# Autodesk Inventor assembly: face
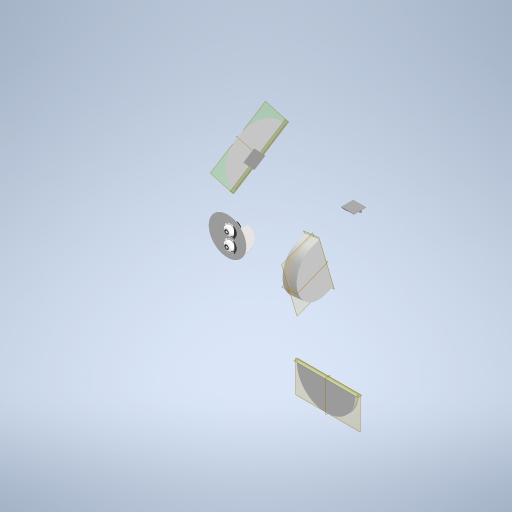
[picture p0: Inventor's stored thumbnail of the model, 512x512]
Saved by Autodesk Inventor 2023.2 (Build 272271030, 271C)
## iProperties
Created: 2024-01-26
Part Number: face
Document SubType Name: Assembly
Designer: I9232
Author: I9232
## Documents named in this file (10)
- D:\!project\fox_n_crow_construction\crow\face\face.iam
- D:\!project\fox_n_crow_construction\crow\face\Сборка глаза вороны.iam
- D:\!project\fox_n_crow_construction\crow\face\Деталь1.ipt
- D:\!project\fox_n_crow_construction\crow\face\Платформа для крыльев лево.ipt
- D:\!project\fox_n_crow_construction\crow\face\Платформа для крыльев право.ipt
- D:\!project\fox_n_crow_construction\crow\face\Сыр.ipt
- D:\!project\fox_n_crow_construction\crow\face\Веер.ipt
- D:\!project\fox_n_crow_construction\crow\face\боковые стороны головы.ipt
- D:\!project\fox_n_crow_construction\crow\face\door_hinge.ipt
- D:\!project\fox_n_crow_construction\crow\face\servoDS3115mg.iam
## Components (10 placed, 9 different names)
1. Сборка глаза вороны:1 [sub-assembly] — Заподлицо:1, Совмещение:5
2. Платформа глаз — Заподлицо:1, Совмещение:2, Совмещение:4, Совмещение:5
3. Платформа для крыльев лево:1
4. Платформа для крыльев право:1 — Жесткий:1
5. Сыр:1
6. Веер:1 — Жесткий:1
7. Веер:2
8. боковые стороны головы:1 — Совмещение:4, Совмещение:6, Совмещение:7, Совмещение:8
9. door_hinge:1 — Совмещение:2
10. servoDS3115mg:1 [sub-assembly] — Совмещение:6, Совмещение:7, Совмещение:8
## Relationships (8: Mate 6, Flush 1, WeldJoint 1)
- Заподлицо:1 [Flush]: Сборка глаза вороны:1 ↔ Платформа глаз
- Жесткий:1 [WeldJoint]: Платформа для крыльев право:1 ↔ Веер:1
- Совмещение:2 [Mate]: Платформа глаз ↔ door_hinge:1
- Совмещение:4 [Mate]: Платформа глаз ↔ боковые стороны головы:1
- Совмещение:5 [Mate]: Сборка глаза вороны:1 ↔ Платформа глаз
- Совмещение:6 [Mate]: боковые стороны головы:1 ↔ servoDS3115mg:1
- Совмещение:7 [Mate]: боковые стороны головы:1 ↔ servoDS3115mg:1
- Совмещение:8 [Mate]: боковые стороны головы:1 ↔ servoDS3115mg:1
